# Autodesk Inventor assembly: Enclosure
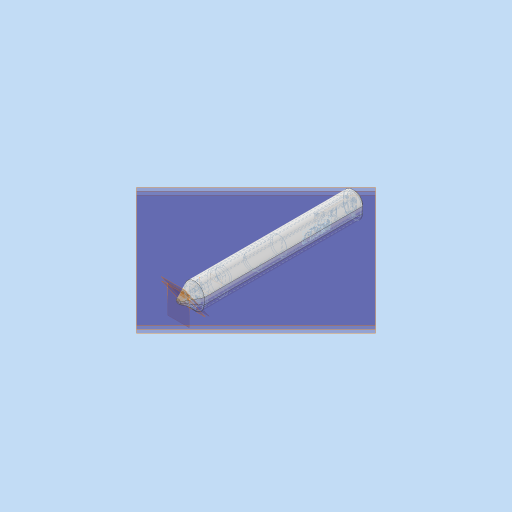
[picture p0: Inventor's stored thumbnail of the model, 512x512]
Saved by Autodesk Inventor 2024 (Build 280153000, 153)
## iProperties
Created: 2025-02-15
Part Number: Enclosure
Document SubType Name: Assembly
Designer: XxPan
Author: XxPan
## Documents named in this file (6)
- C:\Users\XxPan\OneDrive - McMaster University\4OI6\InkSync\case\Enclosure.iam
- C:\Users\XxPan\OneDrive - McMaster University\4OI6\InkSync\case\MCU_PCB.iam
- C:\Users\XxPan\OneDrive - McMaster University\4OI6\InkSync\case\Sensor_PCB.iam
- C:\Users\XxPan\OneDrive - McMaster University\4OI6\InkSync\case\Battery.ipt
- C:\Users\XxPan\OneDrive - McMaster University\4OI6\InkSync\case\Charging_board.ipt
- C:\Users\XxPan\OneDrive - McMaster University\4OI6\InkSync\case\Shell.ipt
## Components (5 placed, 5 different names)
1. MCU_PCB:1 [sub-assembly] — Flush:13, Mate:5, Mate:6
2. Sensor_PCB:1 [sub-assembly] — Flush:5, Flush:6, Flush:7, Flush:8, Flush:11
3. Battery:1 — Mate:1, Flush:1
4. Charging_board:1 — Flush:12, Mate:3, Mate:4, Flush:13, Mate:5, Mate:6
5. Shell:1 — Flush:10, Flush:11, Flush:12, Mate:4
## Relationships (15: Flush 10, Mate 5)
- Mate:1: Battery:1
- Flush:1: Battery:1
- Flush:5: Sensor_PCB:1
- Flush:6: Sensor_PCB:1
- Flush:7: Sensor_PCB:1
- Flush:8: Sensor_PCB:1
- Flush:9 (5 mm)
- Flush:10: Shell:1
- Flush:11 (12 mm): Sensor_PCB:1 ↔ Shell:1
- Flush:12 (0.5 mm): Charging_board:1 ↔ Shell:1
- Mate:3: Charging_board:1
- Mate:4: Charging_board:1 ↔ Shell:1
- Flush:13 (3 mm): MCU_PCB:1 ↔ Charging_board:1
- Mate:5 (1 mm): MCU_PCB:1 ↔ Charging_board:1
- Mate:6: MCU_PCB:1 ↔ Charging_board:1
